# Autodesk Inventor assembly: Assembly1
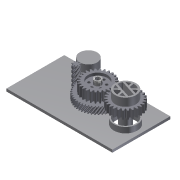
[picture p0: Inventor's stored thumbnail of the model, 180x180]
Saved by Autodesk Inventor 2012 (Build 160160000, 160)
## iProperties
Created: 2017-01-26
Part Number: Assembly1
Document SubType Name: Assembly
Designer: omaro
Author: omaro
## Documents named in this file (12)
- D:\Researches\Gate Motor Gears\_V2\Assembly1.iam
- D:\Researches\Gate Motor Gears\_V2\Casing.ipt
- D:\Researches\Gate Motor Gears\_V2\HelicalGearShaft.ipt
- D:\Researches\Gate Motor Gears\_V2\Assembly1\Design Accelerator\Spur Gears1.iam
- D:\Researches\Gate Motor Gears\_V2\Assembly1\Design Accelerator\Spur Gears2.iam
- D:\Researches\Gate Motor Gears\_V2\HelicalRiser.ipt
- D:\Researches\Gate Motor Gears\_V2\Assembly1\Design Accelerator\Spur Gears3.iam
- D:\Researches\Gate Motor Gears\_V2\DrivingShaft.ipt
- D:\Researches\Gate Motor Gears\_V2\annoyingGear.ipt
- D:\Researches\Gate Motor Gears\_V2\Cover.ipt
- D:\Researches\Gate Motor Gears\_V2\BigGear.iam
- D:\Researches\Gate Motor Gears\_V2\PinionGear.iam
## Components (11 placed, 9 different names)
1. Casing:1 — Mate:1, Mate:2, Mate:5, Mate:6, Mate:8, Mate:11, Mate:12, Flush:2, Flush:3, Mate:27, Mate:29
2. HelicalGearShaft:1 — Mate:1, Mate:2, Mate:7, Mate:21, Mate:23, Mate:25, Mate:26
3. Spur Gears:1 [sub-assembly] — Mate:23, Mate:24
4. Spur Gears:2 [sub-assembly] — Mate:5, Mate:6
5. HelicalRiser:1 — Mate:7, Mate:8, Flush:4
6. Spur Gears:3 [sub-assembly] — Flush:4, Mate:24, Mate:25
7. DrivingShaft:1 — Mate:11, Mate:12, Mate:20
8. annoyingGear:1 — Flush:2
9. Cover:1 — Mate:20, Mate:21, Flush:3, Mate:28
10. BigGear:1 [sub-assembly] — Mate:26, Mate:27, Rotation:1
11. PinionGear:1 [sub-assembly] — Mate:28, Mate:29, Rotation:1
## Relationships (21: Mate 17, Flush 3, RelateRotation 1)
- Mate:1: Casing:1 ↔ HelicalGearShaft:1
- Mate:2 (10 mm): Casing:1 ↔ HelicalGearShaft:1
- Mate:5: Casing:1 ↔ Spur Gears:2
- Mate:6: Casing:1 ↔ Spur Gears:2
- Mate:7: HelicalGearShaft:1 ↔ HelicalRiser:1
- Mate:8: Casing:1 ↔ HelicalRiser:1
- Mate:11: Casing:1 ↔ DrivingShaft:1
- Mate:12 (-6.2 mm): Casing:1 ↔ DrivingShaft:1
- Flush:2: Casing:1 ↔ annoyingGear:1
- Mate:20: DrivingShaft:1 ↔ Cover:1
- Mate:21: HelicalGearShaft:1 ↔ Cover:1
- Flush:3 (-3 mm): Casing:1 ↔ Cover:1
- Flush:4 (3 mm): HelicalRiser:1 ↔ Spur Gears:3
- Mate:23: HelicalGearShaft:1 ↔ Spur Gears:1
- Mate:24: Spur Gears:1 ↔ Spur Gears:3
- Mate:25: HelicalGearShaft:1 ↔ Spur Gears:3
- Mate:26: HelicalGearShaft:1 ↔ BigGear:1
- Mate:27: Casing:1 ↔ BigGear:1
- Mate:28: Cover:1 ↔ PinionGear:1
- Mate:29: Casing:1 ↔ PinionGear:1
- Rotation:1 [RelateRotation] (1 ul): BigGear:1 ↔ PinionGear:1
